# Autodesk Inventor assembly: moisture housing
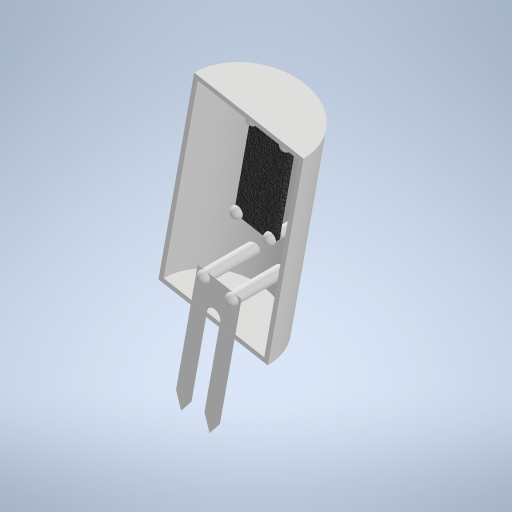
[picture p0: Inventor's stored thumbnail of the model, 512x512]
Saved by Autodesk Inventor 2023 (Build 270158000, 158)
## iProperties
Created: 2023-04-07
Part Number: moisture housing
Document SubType Name: Assembly
Designer: user
Author: user
## Documents named in this file (6)
- C:\Users\user\OneDrive\Desktop\projects\Robotics\smart farm\designs\moisture housing.iam
- C:\Users\user\OneDrive\Desktop\projects\Robotics\smart farm\designs\cover2.ipt
- C:\Users\user\OneDrive\Desktop\projects\Robotics\smart farm\designs\moisture sensor.ipt
- C:\Users\user\OneDrive\Desktop\projects\Robotics\smart farm\designs\screws.ipt
- C:\Users\user\OneDrive\Desktop\projects\Robotics\smart farm\designs\arduino nano screw ports.ipt
- C:\Users\user\OneDrive\Desktop\projects\Robotics\smart farm\designs\board screws.ipt
## Components (9 placed, 5 different names)
1. cover2:1 — Mate:1, Mate:2, Cylindrical:1, Rotation:1, Cylindrical:2, Mate:3, Mate:4, Mate:5, Mate:6
2. moisture sensor:1 — Mate:1, Mate:2
3. screws:1 — Cylindrical:1
4. screws:2 — Rotation:1, Cylindrical:2
5. arduino nano screw ports:1 — Mate:3, Mate:4, Mate:5, Mate:6, Cylindrical:3, Cylindrical:4, Cylindrical:5, Cylindrical:6
6. board screws:1 — Cylindrical:4
7. board screws:2 — Cylindrical:3
8. board screws:3 — Cylindrical:5
9. board screws:4 — Cylindrical:6
## Relationships (13: Mate 6, CylindricalJoint 6, RelateRotation 1)
- Mate:1: cover2:1 ↔ moisture sensor:1
- Mate:2: cover2:1 ↔ moisture sensor:1
- Cylindrical:1: cover2:1 ↔ screws:1
- Rotation:1 [RelateRotation] (1 ul): cover2:1 ↔ screws:2
- Cylindrical:2: cover2:1 ↔ screws:2
- Mate:3: cover2:1 ↔ arduino nano screw ports:1
- Mate:4: cover2:1 ↔ arduino nano screw ports:1
- Mate:5: cover2:1 ↔ arduino nano screw ports:1
- Mate:6: cover2:1 ↔ arduino nano screw ports:1
- Cylindrical:3: arduino nano screw ports:1 ↔ board screws:2
- Cylindrical:4: arduino nano screw ports:1 ↔ board screws:1
- Cylindrical:5: arduino nano screw ports:1 ↔ board screws:3
- Cylindrical:6: arduino nano screw ports:1 ↔ board screws:4
